# Autodesk Inventor assembly: Ra-Manager_Montagem_Controller
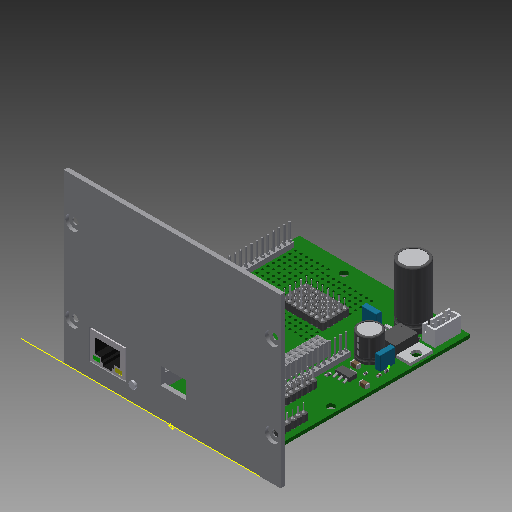
[picture p0: Inventor's stored thumbnail of the model, 512x512]
Saved by Autodesk Inventor 2019.4 (Build 234330000, 330)
## iProperties
Created: 2020-03-12
Part Number: Ra-Manager_Montagem_Controller
Material: Genérico
Document SubType Name: Assembly
Designer: caio.santos
Author: caio.santos
## Documents named in this file (4)
- C:\Users\caiom\Desktop\Ra-Manager_Mecanica\Ra-Manager_Montagem_Controller.iam
- C:\Users\caiom\Desktop\Ra-Manager_Mecanica\Ra-Manager_Painel-Placas.ipt
- C:\Users\caiom\Desktop\Ra-Manager_Mecanica\Ra-Manager_Light_Pipe.ipt
- C:\Users\caiom\Desktop\Ra-Manager_Mecanica\ExportSTEP\RA-Manager_Controller.ipt
## Components (3 placed, 3 different names)
1. Ra-Manager_Painel-Placas:1 — Coincidência:2, Coincidência:3, Coincidência:5, Coincidência:8, Coincidência:9, Alinhamento:1, Alinhamento:2, Coincidência:10
2. RA-Manager_Controller:2 — Alinhamento:1, Alinhamento:2, Coincidência:10
3. Ra-Manager_Light_Pipe:1 — Coincidência:8, Coincidência:9
## Relationships (9: Mate 7, Flush 2)
- Coincidência:2 [Mate]: Ra-Manager_Painel-Placas:1
- Coincidência:3 [Mate]: Ra-Manager_Painel-Placas:1
- Coincidência:5 [Mate]: Ra-Manager_Painel-Placas:1
- Coincidência:6 [Mate]
- Coincidência:8 [Mate]: Ra-Manager_Painel-Placas:1 ↔ Ra-Manager_Light_Pipe:1
- Coincidência:9 [Mate]: Ra-Manager_Painel-Placas:1 ↔ Ra-Manager_Light_Pipe:1
- Alinhamento:1 [Flush] (5.75 mm): Ra-Manager_Painel-Placas:1 ↔ RA-Manager_Controller:2
- Alinhamento:2 [Flush] (10.7625 mm): Ra-Manager_Painel-Placas:1 ↔ RA-Manager_Controller:2
- Coincidência:10 [Mate] (2.75 mm): Ra-Manager_Painel-Placas:1 ↔ RA-Manager_Controller:2
